# Autodesk Inventor assembly: Tower
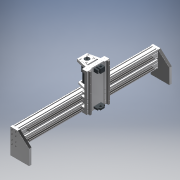
[picture p0: Inventor's stored thumbnail of the model, 180x180]
Saved by Autodesk Inventor 2019 (Build 230136000, 136)
## iProperties
Created: 2021-05-10
Part Number: Tower
Document SubType Name: Assembly
Designer: Lenovo
Author: Lenovo
## Documents named in this file (28)
- C:\Users\Michael Sumper\OneDrive\Documents\Inventor\Portalfräse Devil'sCNC\Tower.iam
- C:\Users\Michael Sumper\OneDrive\Documents\Inventor\Portalfräse Devil'sCNC\60x60x1100 Profil.ipt
- C:\Users\Michael Sumper\OneDrive\Documents\Inventor\Portalfräse Devil'sCNC\1000mmFührung.ipt
- C:\Users\Michael Sumper\OneDrive\Documents\Inventor\Portalfräse Devil'sCNC\Führungswagen.ipt
- C:\Users\Michael Sumper\OneDrive\Documents\Inventor\Portalfräse Devil'sCNC\Kreuzplatte.ipt
- C:\Users\Michael Sumper\OneDrive\Documents\Inventor\Portalfräse Devil'sCNC\Tower\Konstruktions-Assistent\Schraubenverbindung18.iam
- C:\Users\Michael Sumper\OneDrive\Documents\Inventor\Portalfräse Devil'sCNC\Linearführung.ipt
- C:\Users\Michael Sumper\OneDrive\Documents\Inventor\Portalfräse Devil'sCNC\Tower\Konstruktions-Assistent\Schraubenverbindung19.iam
- C:\Users\Michael Sumper\OneDrive\Documents\Inventor\Portalfräse Devil'sCNC\Tower\Konstruktions-Assistent\Schraubenverbindung20.iam
- C:\Users\Michael Sumper\OneDrive\Documents\Inventor\Portalfräse Devil'sCNC\Loslager.ipt
- C:\Users\Michael Sumper\OneDrive\Documents\Inventor\Portalfräse Devil'sCNC\Festlager.ipt
- C:\Users\Michael Sumper\OneDrive\Documents\Inventor\Portalfräse Devil'sCNC\Tower\Konstruktions-Assistent\Schraubenverbindung21.iam
- C:\Users\Michael Sumper\OneDrive\Documents\Inventor\Portalfräse Devil'sCNC\Tower\Konstruktions-Assistent\Schraubenverbindung23.iam
- C:\Users\Michael Sumper\OneDrive\Documents\Inventor\Portalfräse Devil'sCNC\Y-Motorhalter.ipt
- C:\Users\Michael Sumper\OneDrive\Documents\Inventor\Portalfräse Devil'sCNC\Z-Motoraufnahme.ipt
- C:\Users\Michael Sumper\OneDrive\Documents\Inventor\Portalfräse Devil'sCNC\Z-Motorhalter.ipt
- C:\Users\Michael Sumper\OneDrive\Documents\Inventor\Portalfräse Devil'sCNC\NEMA23.ipt
- C:\Users\Michael Sumper\OneDrive\Documents\Inventor\Portalfräse Devil'sCNC\Tower\Konstruktions-Assistent\Schraubenverbindung22.iam
- C:\Users\Michael Sumper\OneDrive\Documents\Inventor\Portalfräse Devil'sCNC\Tower\Konstruktions-Assistent\Schraubenverbindung24.iam
- C:\Users\Michael Sumper\OneDrive\Documents\Inventor\Portalfräse Devil'sCNC\Tower\Konstruktions-Assistent\Schraubenverbindung25.iam
- C:\Users\Michael Sumper\OneDrive\Documents\Inventor\Portalfräse Devil'sCNC\Tower\Konstruktions-Assistent\Schraubenverbindung26.iam
- C:\Users\Michael Sumper\OneDrive\Documents\Inventor\Portalfräse Devil'sCNC\Tower\Konstruktions-Assistent\Schraubenverbindung28.iam
- C:\Users\Michael Sumper\OneDrive\Documents\Inventor\Portalfräse Devil'sCNC\Tower\Konstruktions-Assistent\Schraubenverbindung29.iam
- C:\Users\Michael Sumper\OneDrive\Documents\Inventor\Portalfräse Devil'sCNC\Tower\Konstruktions-Assistent\Schraubenverbindung30.iam
- C:\Users\Michael Sumper\OneDrive\Documents\Inventor\Portalfräse Devil'sCNC\Tower\Konstruktions-Assistent\Schraubenverbindung31.iam
- C:\Users\Michael Sumper\OneDrive\Documents\Inventor\Portalfräse Devil'sCNC\Portalwange.ipt
- C:\Users\Michael Sumper\OneDrive\Documents\Inventor\Portalfräse Devil'sCNC\Tower\Konstruktions-Assistent\Schraubenverbindung27.iam
- C:\Users\Michael Sumper\OneDrive\Documents\Inventor\Portalfräse Devil'sCNC\Tower\Konstruktions-Assistent\Schraubenverbindung32.iam
## Components (35 placed, 13 different names)
1. 60x60x1100 Profil:1 — Passend:1, Fluchtend:1, Fluchtend:2, Passend:2, Fluchtend:3, Fluchtend:4, Passend:68, Passend:69, Passend:71, Passend:72
2. 60x60x1100 Profil:2 — Passend:1, Fluchtend:1, Fluchtend:2, Passend:3, Fluchtend:5, Fluchtend:6, Passend:67, Passend:70
3. Führung:1 — Passend:3, Fluchtend:5, Fluchtend:6, Zylindrisch:1, Zylindrisch:2
4. Führung:2 — Passend:2, Fluchtend:3, Fluchtend:4, Zylindrisch:3, Zylindrisch:4
5. Führungswagen:1 — Zylindrisch:4, Passend:5
6. Führungswagen:2 — Zylindrisch:3, Passend:8
7. Führungswagen:3 — Zylindrisch:1, Passend:7
8. Führungswagen:4 — Zylindrisch:2, Passend:4, Passend:6
9. Kreuzplatte:1 — Passend:4, Passend:5, Passend:6, Passend:7, Passend:8, Passend:9, Passend:10, Zylindrisch:5, Zylindrisch:6, Passend:11, Passend:12, Passend:13, Passend:14, Passend:15, Passend:16, Passend:21, Passend:22, Passend:23, Passend:24, Passend:25, Passend:26, Passend:31, Passend:32, Passend:33, Passend:34, Passend:35, Passend:36, Passend:49, Passend:50
10. Schraubenverbindung:1 [sub-assembly] — Passend:9, Passend:10, Zylindrisch:5, Zylindrisch:6
11. Linearführung:1 — Passend:11, Passend:12, Passend:13, Passend:17, Passend:18, Zylindrisch:7, Zylindrisch:8
12. Linearführung:2 — Passend:14, Passend:15, Passend:16, Passend:19, Passend:20, Zylindrisch:9, Zylindrisch:10
13. Schraubenverbindung:2 [sub-assembly] — Passend:17, Passend:18, Zylindrisch:7, Zylindrisch:8
14. Schraubenverbindung:3 [sub-assembly] — Passend:19, Passend:20, Zylindrisch:9, Zylindrisch:10
15. Loslager:1 — Passend:21, Passend:22, Passend:23, Passend:29, Passend:30, Passend:44
16. Festlager:1 — Passend:24, Passend:25, Passend:26, Passend:27, Passend:28, Passend:43
17. Schraubenverbindung:4 [sub-assembly] — Passend:27, Passend:28, Passend:43
18. Schraubenverbindung:5 [sub-assembly] — Passend:29, Passend:30, Passend:44
19. Y-Motorhalter:1 — Passend:34, Passend:35, Passend:36, Passend:37, Passend:38, Passend:39, Passend:47, Passend:48
20. Z-Motoraufnahme:1 — Verschiebbar:1, Passend:40, Passend:41, Passend:42, Passend:79, Passend:81, Passend:83, Passend:85
21. Z-Motorhalter:1 — Passend:31, Passend:32, Passend:33, Verschiebbar:1, Passend:45, Passend:46, Passend:80, Passend:82, Passend:84, Passend:86
22. NEMA23:1 — Passend:37, Passend:38, Passend:39, Passend:53, Passend:54, Passend:55
23. NEMA23:2 — Passend:40, Passend:41, Passend:42, Passend:56, Passend:87, Passend:88
24. Schraubenverbindung:6 [sub-assembly] — Passend:45, Passend:46, Passend:50
25. Schraubenverbindung:7 [sub-assembly] — Passend:47, Passend:48, Passend:49
26. Schraubenverbindung:8 [sub-assembly] — Passend:56, Passend:87, Passend:88
27. Schraubenverbindung:9 [sub-assembly] — Passend:53, Passend:54, Passend:55
28. Schraubenverbindung:11 [sub-assembly] — Passend:79, Passend:80
29. Schraubenverbindung:12 [sub-assembly] — Passend:81, Passend:82
30. Schraubenverbindung:13 [sub-assembly] — Passend:83, Passend:84
31. Schraubenverbindung:14 [sub-assembly] — Passend:85, Passend:86
32. Portalwange:1 — Passend:67, Passend:68, Passend:69, Passend:73, Passend:74, Passend:78
33. Portalwange:2 — Passend:70, Passend:71, Passend:72, Passend:75, Passend:76, Passend:77
34. Schraubenverbindung:15 [sub-assembly] — Passend:73, Passend:74, Passend:78
35. Schraubenverbindung:16 [sub-assembly] — Passend:75, Passend:76, Passend:77
## Relationships (93: Mate 76, CylindricalJoint 10, Flush 6, TranslationJoint 1)
- Passend:1 [Mate] (10 mm): 60x60x1100 Profil:1 ↔ 60x60x1100 Profil:2
- Fluchtend:1 [Flush]: 60x60x1100 Profil:1 ↔ 60x60x1100 Profil:2
- Fluchtend:2 [Flush]: 60x60x1100 Profil:1 ↔ 60x60x1100 Profil:2
- Passend:2 [Mate]: 60x60x1100 Profil:1 ↔ Führung:2
- Fluchtend:3 [Flush]: 60x60x1100 Profil:1 ↔ Führung:2
- Fluchtend:4 [Flush] (50 mm): 60x60x1100 Profil:1 ↔ Führung:2
- Passend:3 [Mate]: 60x60x1100 Profil:2 ↔ Führung:1
- Fluchtend:5 [Flush]: 60x60x1100 Profil:2 ↔ Führung:1
- Fluchtend:6 [Flush] (50 mm): 60x60x1100 Profil:2 ↔ Führung:1
- Zylindrisch:1 [CylindricalJoint]: Führung:1 ↔ Führungswagen:3
- Zylindrisch:2 [CylindricalJoint]: Führung:1 ↔ Führungswagen:4
- Zylindrisch:3 [CylindricalJoint]: Führung:2 ↔ Führungswagen:2
- Zylindrisch:4 [CylindricalJoint]: Führung:2 ↔ Führungswagen:1
- Passend:4 [Mate]: Führungswagen:4 ↔ Kreuzplatte:1
- Passend:5 [Mate]: Führungswagen:1 ↔ Kreuzplatte:1
- Passend:6 [Mate]: Führungswagen:4 ↔ Kreuzplatte:1
- Passend:7 [Mate]: Führungswagen:3 ↔ Kreuzplatte:1
- Passend:8 [Mate]: Führungswagen:2 ↔ Kreuzplatte:1
- Passend:9 [Mate]: Kreuzplatte:1 ↔ Schraubenverbindung:1
- Passend:10 [Mate]: Kreuzplatte:1 ↔ Schraubenverbindung:1
- Zylindrisch:5 [CylindricalJoint]: Kreuzplatte:1 ↔ Schraubenverbindung:1
- Zylindrisch:6 [CylindricalJoint]: Kreuzplatte:1 ↔ Schraubenverbindung:1
- Passend:11 [Mate]: Kreuzplatte:1 ↔ Linearführung:1
- Passend:12 [Mate]: Kreuzplatte:1 ↔ Linearführung:1
- Passend:13 [Mate]: Kreuzplatte:1 ↔ Linearführung:1
- Passend:14 [Mate]: Kreuzplatte:1 ↔ Linearführung:2
- Passend:15 [Mate]: Kreuzplatte:1 ↔ Linearführung:2
- Passend:16 [Mate]: Kreuzplatte:1 ↔ Linearführung:2
- Passend:17 [Mate]: Linearführung:1 ↔ Schraubenverbindung:2
- Passend:18 [Mate]: Linearführung:1 ↔ Schraubenverbindung:2
- Passend:19 [Mate]: Linearführung:2 ↔ Schraubenverbindung:3
- Passend:20 [Mate]: Linearführung:2 ↔ Schraubenverbindung:3
- Zylindrisch:7 [CylindricalJoint]: Linearführung:1 ↔ Schraubenverbindung:2
- Zylindrisch:8 [CylindricalJoint]: Linearführung:1 ↔ Schraubenverbindung:2
- Zylindrisch:9 [CylindricalJoint]: Linearführung:2 ↔ Schraubenverbindung:3
- Zylindrisch:10 [CylindricalJoint]: Linearführung:2 ↔ Schraubenverbindung:3
- Passend:21 [Mate]: Kreuzplatte:1 ↔ Loslager:1
- Passend:22 [Mate]: Kreuzplatte:1 ↔ Loslager:1
- Passend:23 [Mate]: Kreuzplatte:1 ↔ Loslager:1
- Passend:24 [Mate]: Kreuzplatte:1 ↔ Festlager:1
- Passend:25 [Mate]: Kreuzplatte:1 ↔ Festlager:1
- Passend:26 [Mate]: Kreuzplatte:1 ↔ Festlager:1
- Passend:27 [Mate]: Festlager:1 ↔ Schraubenverbindung:4
- Passend:28 [Mate]: Festlager:1 ↔ Schraubenverbindung:4
- Passend:29 [Mate]: Loslager:1 ↔ Schraubenverbindung:5
- Passend:30 [Mate]: Loslager:1 ↔ Schraubenverbindung:5
- Passend:31 [Mate]: Kreuzplatte:1 ↔ Z-Motorhalter:1
- Passend:32 [Mate]: Kreuzplatte:1 ↔ Z-Motorhalter:1
- Passend:33 [Mate]: Kreuzplatte:1 ↔ Z-Motorhalter:1
- Passend:34 [Mate]: Kreuzplatte:1 ↔ Y-Motorhalter:1
- Passend:35 [Mate]: Kreuzplatte:1 ↔ Y-Motorhalter:1
- Passend:36 [Mate]: Kreuzplatte:1 ↔ Y-Motorhalter:1
- Verschiebbar:1 [TranslationJoint]: Z-Motoraufnahme:1 ↔ Z-Motorhalter:1
- Passend:37 [Mate]: Y-Motorhalter:1 ↔ NEMA23:1
- Passend:38 [Mate]: Y-Motorhalter:1 ↔ NEMA23:1
- Passend:39 [Mate]: Y-Motorhalter:1 ↔ NEMA23:1
- Passend:40 [Mate]: Z-Motoraufnahme:1 ↔ NEMA23:2
- Passend:41 [Mate]: Z-Motoraufnahme:1 ↔ NEMA23:2
- Passend:42 [Mate]: Z-Motoraufnahme:1 ↔ NEMA23:2
- Passend:43 [Mate]: Festlager:1 ↔ Schraubenverbindung:4
- Passend:44 [Mate]: Loslager:1 ↔ Schraubenverbindung:5
- Passend:45 [Mate]: Z-Motorhalter:1 ↔ Schraubenverbindung:6
- Passend:46 [Mate]: Z-Motorhalter:1 ↔ Schraubenverbindung:6
- Passend:47 [Mate]: Y-Motorhalter:1 ↔ Schraubenverbindung:7
- Passend:48 [Mate]: Y-Motorhalter:1 ↔ Schraubenverbindung:7
- Passend:49 [Mate]: Kreuzplatte:1 ↔ Schraubenverbindung:7
- Passend:50 [Mate]: Kreuzplatte:1 ↔ Schraubenverbindung:6
- Passend:53 [Mate]: NEMA23:1 ↔ Schraubenverbindung:9
- Passend:54 [Mate]: NEMA23:1 ↔ Schraubenverbindung:9
- Passend:55 [Mate]: NEMA23:1 ↔ Schraubenverbindung:9
- Passend:56 [Mate]: NEMA23:2 ↔ Schraubenverbindung:8
- Passend:67 [Mate]: 60x60x1100 Profil:2 ↔ Portalwange:1
- Passend:68 [Mate]: 60x60x1100 Profil:1 ↔ Portalwange:1
- Passend:69 [Mate]: 60x60x1100 Profil:1 ↔ Portalwange:1
- Passend:70 [Mate]: 60x60x1100 Profil:2 ↔ Portalwange:2
- Passend:71 [Mate]: 60x60x1100 Profil:1 ↔ Portalwange:2
- Passend:72 [Mate]: 60x60x1100 Profil:1 ↔ Portalwange:2
- Passend:73 [Mate]: Portalwange:1 ↔ Schraubenverbindung:15
- Passend:74 [Mate]: Portalwange:1 ↔ Schraubenverbindung:15
- Passend:75 [Mate]: Portalwange:2 ↔ Schraubenverbindung:16
- Passend:76 [Mate]: Portalwange:2 ↔ Schraubenverbindung:16
- Passend:77 [Mate]: Portalwange:2 ↔ Schraubenverbindung:16
- Passend:78 [Mate]: Portalwange:1 ↔ Schraubenverbindung:15
- Passend:79 [Mate]: Z-Motoraufnahme:1 ↔ Schraubenverbindung:11
- Passend:80 [Mate]: Z-Motorhalter:1 ↔ Schraubenverbindung:11
- Passend:81 [Mate]: Z-Motoraufnahme:1 ↔ Schraubenverbindung:12
- Passend:82 [Mate]: Z-Motorhalter:1 ↔ Schraubenverbindung:12
- Passend:83 [Mate]: Z-Motoraufnahme:1 ↔ Schraubenverbindung:13
- Passend:84 [Mate]: Z-Motorhalter:1 ↔ Schraubenverbindung:13
- Passend:85 [Mate]: Z-Motoraufnahme:1 ↔ Schraubenverbindung:14
- Passend:86 [Mate]: Z-Motorhalter:1 ↔ Schraubenverbindung:14
- Passend:87 [Mate]: NEMA23:2 ↔ Schraubenverbindung:8
- Passend:88 [Mate]: NEMA23:2 ↔ Schraubenverbindung:8
